# Autodesk Inventor assembly: holderStack
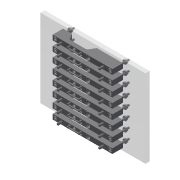
[picture p0: Inventor's stored thumbnail of the model, 180x180]
Saved by Autodesk Inventor 2018 (Build 220112000, 112)
## iProperties
Created: 2017-05-11
Part Number: holderStack
Document SubType Name: Assembly
Designer: sawaiz
Author: sawaiz
## Documents named in this file (6)
- C:\Users\sawaiz\OneDrive\projects\sPhenixTileTestStand\sipmHolder\holderStack.iam
- C:\Users\sawaiz\OneDrive\projects\sPhenixTileTestStand\sipmHolder\holderStack.ipt
- C:\Users\sawaiz\OneDrive\projects\sPhenixTileTestStand\sipmHolder\sipmHolderLonger.ipt
- C:\Users\sawaiz\OneDrive\projects\sPhenixTileTestStand\hardware\m2.5x25.ipt
- C:\Users\sawaiz\OneDrive\projects\sPhenixTileTestStand\hardware\m2.5washer.ipt
- C:\Users\sawaiz\OneDrive\projects\sPhenixTileTestStand\hardware\m2.5nut.ipt
## Components (57 placed, 5 different names)
1. holderStack:1 — Mate:1, Mate:2, Mate:3, Mate:9
2. sipmHolderLonger:1 — Mate:1, Mate:2, Mate:3, Mate:4, Mate:5, Mate:6
3. m2.5x25:1 — Mate:4, Mate:5, Flush:1, Mate:8, Mate:11
4. m2.5x25:2 — Mate:6, Flush:1, Mate:7, Mate:10
5. m2.5washer:1 — Mate:8, Flush:2
6. m2.5washer:2 — Mate:7, Flush:2, Mate:9, Mate:12
7. m2.5nut:1 — Flush:3, Flush:4, Mate:10, Mate:12
8. m2.5nut:2 — Flush:3, Flush:4, Mate:11
9. sipmHolderLonger:2
10. m2.5x25:3
11. m2.5x25:4
12. m2.5washer:3
13. m2.5washer:4
14. m2.5nut:3
15. m2.5nut:4
16. sipmHolderLonger:3
17. m2.5x25:5
18. m2.5x25:6
19. m2.5washer:5
20. m2.5washer:6
21. m2.5nut:5
22. m2.5nut:6
23. sipmHolderLonger:4
24. m2.5x25:7
25. m2.5x25:8
26. m2.5washer:7
27. m2.5washer:8
28. m2.5nut:7
29. m2.5nut:8
30. sipmHolderLonger:5
31. m2.5x25:9
32. m2.5x25:10
33. m2.5washer:9
34. m2.5washer:10
35. m2.5nut:9
36. m2.5nut:10
37. sipmHolderLonger:6
38. m2.5x25:11
39. m2.5x25:12
40. m2.5washer:11
41. m2.5washer:12
42. m2.5nut:11
43. m2.5nut:12
44. sipmHolderLonger:7
45. m2.5x25:13
46. m2.5x25:14
47. m2.5washer:13
48. m2.5washer:14
49. m2.5nut:13
50. m2.5nut:14
51. sipmHolderLonger:8
52. m2.5x25:15
53. m2.5x25:16
54. m2.5washer:15
55. m2.5washer:16
56. m2.5nut:15
57. m2.5nut:16
## Component patterns: (8 elements, first: sipmHolderLonger:1 + m2.5x25:1 + m2.5x25:2 + m2.5washer:1 + m2.5washer:2 + m2.5nut:1 + m2.5nut:2)
## Relationships (16: Mate 12, Flush 4)
- Mate:1: holderStack:1 ↔ sipmHolderLonger:1
- Mate:2: holderStack:1 ↔ sipmHolderLonger:1
- Mate:3: holderStack:1 ↔ sipmHolderLonger:1
- Mate:4: sipmHolderLonger:1 ↔ m2.5x25:1
- Mate:5: sipmHolderLonger:1 ↔ m2.5x25:1
- Mate:6: sipmHolderLonger:1 ↔ m2.5x25:2
- Flush:1: m2.5x25:1 ↔ m2.5x25:2
- Mate:7: m2.5x25:2 ↔ m2.5washer:2
- Mate:8: m2.5x25:1 ↔ m2.5washer:1
- Flush:2: m2.5washer:1 ↔ m2.5washer:2
- Mate:9: holderStack:1 ↔ m2.5washer:2
- Flush:3: m2.5nut:1 ↔ m2.5nut:2
- Flush:4: m2.5nut:1 ↔ m2.5nut:2
- Mate:10: m2.5x25:2 ↔ m2.5nut:1
- Mate:11: m2.5x25:1 ↔ m2.5nut:2
- Mate:12: m2.5washer:2 ↔ m2.5nut:1
